# Autodesk Inventor assembly: SCSWA6-8
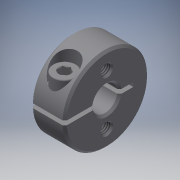
[picture p0: Inventor's stored thumbnail of the model, 180x180]
Saved by Autodesk Inventor 2019 (Build 230136000, 136)
## iProperties
Category: PARTsolutions
Company: MISUMI
Created: 2024-10-12
Part Number: SCSWA6-8
Catalog Web Link: www.cadenas.de
Description: SCSW, PSCSW, SSCSW, SCSWA, SCSWAW-Set Collars - Slit 2 Hole/2 Tap - Standard Type - 2 Tap Type
Vendor: MISUMI
Document SubType Name: Assembly
Designer: psAdmin
Manufacturer: MISUMI
Mass: 2.06471 g
Surface Area: 17.3178 cm^2
Volume: 2.06471 cm^3
Density: 1 g/cm^3
Title: SCSWA6-8
Author: Cadenas PARTsolutions
Comments: Set Collars - Slit 2 Hole/2 Tap - Standard Type - 2 Tap Type
PSOL_IDENT_0: {$CADENAS_DATA/23d-libs/misumi/metric/03_set_collars/scsw_asmtab.prj},209 {VTYP=3D},{STYP=ASSTAB},{N
PSOL_IDENT_1: B=SCSWA6-8},{LINA=SCSWA6-8},{NN=SCSW, PSCSW, SSCSW, SCSWA, SCSWAW},{DATE=30.11.2021 05:42:05},{GEOMD
PSOL_IDENT_2: ATE=15.09.2021 06:02:54},{VERSION=},{LINEID=220},{WBVAR=MAT,ST,BS},{WBNUMERIC=BS}  {NB=SCSWA6-8},{LI
PSOL_IDENT_3: NA=SCSWA6-8},{KT=DUMMY},{PN=SCSWA6-8},{TYPE=SCSWA},{MAT=2017},{MATA='1045','S45C Equivalent','304','
PSOL_IDENT_4: SUS304 Equivalent','2017','2017 Aluminum Alloy'},{ST=-},{AC=Hexagon Socket Head Set Screw 1 Pc. (304
PSOL_IDENT_5: Stainless Steel) },{D=6},{BS=8},{B1=8,10},{D1=20},{M=M3},{THMD=3},{THDMIN=2.459},{ST0='-','-','Clea
PSOL_IDENT_6: r Anodize','Clear Anodize'},{DD=3.4},{R=3.00},{W=1.0},{X=6.0},{Y=4.0},{Z=6~6.5},{S=3.5},{P=12},{C=0.
PSOL_IDENT_7: 5},{L=10},{M1=M3},{ZZ=6.25},{THMD1=3},{THDMIN1=2.459},{PPATH=scsw_templ.prj}
NB: SCSWA6-8
NN: SCSW, PSCSW, SSCSW, SCSWA, SCSWAW
NT: Set Collars - Slit 2 Hole/2 Tap - Standard Type - 2 Tap Type
NBSYN: $PN.
LINA: SCSWA6-8
CATALOG: Misumi
PN: SCSWA6-8
MAT: 2017 Aluminum Alloy
ST: -
AC: Hexagon Socket Head Set Screw 1 Pc. (304 Stainless Steel)
D: 6
BS: 8
D1: 20
M: M3
DD: 3.4
R: 3
W: 1
X: 6
Y: 4
Z: 6~6.5
S: 3.5
P: 12
M1: M3
SUPPLIER: MISUMI
ARTICLENO: SCSWA6-8
BOMINFO: SCSWA6-8
CREATOR: CADENAS GmbH
## Documents named in this file (3)
- e:\temp\worker_COMMON_53\temp\tmp_6864_178_mWhRI\format_0\SCSWA6-8.iam
- e:\temp\worker_COMMON_53\temp\tmp_6864_178_mWhRI\format_0\SCSWA6-8b.ipt
- e:\temp\worker_COMMON_53\temp\tmp_6864_178_mWhRI\format_0\Slotted head cap screw ISO 4762 - M3x10.ipt
## Components (2 placed, 2 different names)
1. SCSWA6-8b:1 — body_screw_Z@1 <-> IP1_Z@2
2. Slotted head cap screw ISO 4762 - M3x10:1 — body_screw_Z@1 <-> IP1_Z@2
## Relationships (1: Mate 1)
- body_screw_Z@1 <-> IP1_Z@2 [Mate]: SCSWA6-8b:1 ↔ Slotted head cap screw ISO 4762 - M3x10:1
